# Autodesk Inventor assembly: span
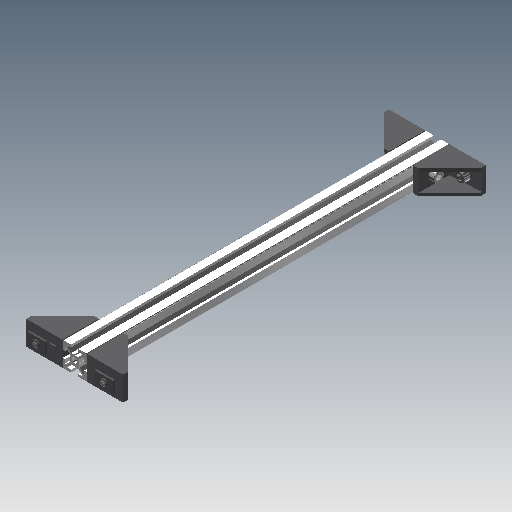
[picture p0: Inventor's stored thumbnail of the model, 512x512]
Saved by Autodesk Inventor 2018 (Build 220112000, 112)
## iProperties
Created: 2017-04-19
Part Number: span
Document SubType Name: Assembly
Designer: sawaiz
Author: sawaiz
## Documents named in this file (3)
- C:\Users\sawaiz\OneDrive\projects\sPhenixTileTestStand\frame\span.iam
- C:\Users\sawaiz\OneDrive\projects\sPhenixTileTestStand\frame\hfs5-2020Width.ipt
- C:\Users\sawaiz\OneDrive\projects\sPhenixTileTestStand\hardware\angleBracket.iam
## Components (5 placed, 2 different names)
1. hfs5-2020Width:1 — Flush:1, Flush:2, Flush:3, Flush:4, Flush:6, Flush:8, Mate:1, Mate:2, Mate:3, Mate:4
2. angleBracket:1 [sub-assembly] — Flush:1, Flush:5, Flush:6, Mate:4, Symmetry:3
3. angleBracket:2 [sub-assembly] — Flush:2, Flush:5, Mate:3, Symmetry:2, Symmetry:3
4. angleBracket:3 [sub-assembly] — Flush:4, Flush:7, Flush:8, Mate:1, Symmetry:1, Symmetry:2
5. angleBracket:4 [sub-assembly] — Flush:3, Flush:7, Mate:2, Symmetry:1
## Relationships (15: Flush 8, Mate 4, Symmetry 3)
- Flush:1: hfs5-2020Width:1 ↔ angleBracket:1
- Flush:2: hfs5-2020Width:1 ↔ angleBracket:2
- Flush:3: hfs5-2020Width:1 ↔ angleBracket:4
- Flush:4: hfs5-2020Width:1 ↔ angleBracket:3
- Flush:5: angleBracket:1 ↔ angleBracket:2
- Flush:6: hfs5-2020Width:1 ↔ angleBracket:1
- Flush:7: angleBracket:3 ↔ angleBracket:4
- Flush:8: hfs5-2020Width:1 ↔ angleBracket:3
- Mate:1: hfs5-2020Width:1 ↔ angleBracket:3
- Mate:2: hfs5-2020Width:1 ↔ angleBracket:4
- Mate:3: hfs5-2020Width:1 ↔ angleBracket:2
- Mate:4: hfs5-2020Width:1 ↔ angleBracket:1
- Symmetry:1: angleBracket:3 ↔ angleBracket:4
- Symmetry:2: angleBracket:2 ↔ angleBracket:3
- Symmetry:3: angleBracket:1 ↔ angleBracket:2
